# Autodesk Inventor assembly: AM14U Wide Dan's 1-7 edits
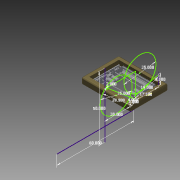
[picture p0: Inventor's stored thumbnail of the model, 180x180]
Saved by Autodesk Inventor 2014 (Build 180170000, 170)
## iProperties
Created: 2014-01-06
Part Number: AM14U Wide Dan's 1-7 edits
Document SubType Name: Assembly
Designer: robotics
Author: robotics
## Documents named in this file (4)
- C:\Users\pc\Dropbox\Cad 2014 Build Season\Robot 2014\Kitbot\AM14U Wide Dan's 1-7 edits.iam
- C:\Users\pc\Dropbox\Cad 2014 Build Season\Robot 2014\Imported Components\AM14U Long and AM14U Wide\AM14U Wide Half.iam
- C:\Users\pc\Dropbox\Cad 2014 Build Season\Robot 2014\Kitbot\bumpers.ipt
- C:\Users\pc\Dropbox\Cad 2014 Build Season\Robot 2014\Kitbot\daball.ipt
## Components (4 placed, 4 different names)
1. AM14U Wide Half_3 [sub-assembly] — Mate:3, Mate:4, Flush:1, Flush:2
2. AM14U Wide Half_4 [sub-assembly] — Mate:1, Mate:2, Flush:1
3. bumpers:1 — Mate:1, Mate:2, Mate:3, Mate:4, Flush:2
4. daball:1
## Relationships (6: Mate 4, Flush 2)
- Mate:1: AM14U Wide Half_4 ↔ bumpers:1
- Mate:2: AM14U Wide Half_4 ↔ bumpers:1
- Mate:3: AM14U Wide Half_3 ↔ bumpers:1
- Mate:4: AM14U Wide Half_3 ↔ bumpers:1
- Flush:1: AM14U Wide Half_3 ↔ AM14U Wide Half_4
- Flush:2 (25.4 mm): AM14U Wide Half_3 ↔ bumpers:1
